# Autodesk Inventor assembly: Walls--Basement
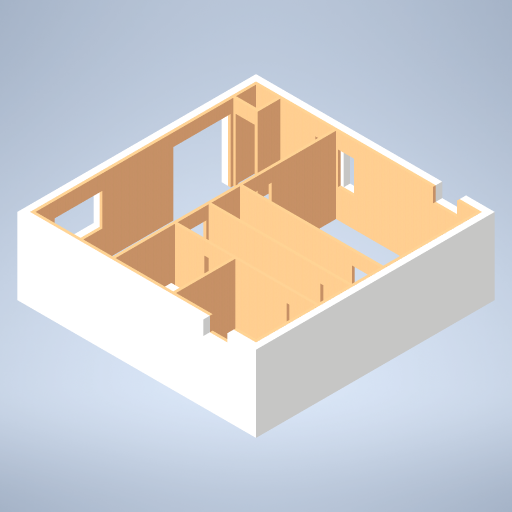
[picture p0: Inventor's stored thumbnail of the model, 512x512]
Saved by Autodesk Inventor 2024 (Build 280153000, 153)
## iProperties
Created: 2023-05-13
Part Number: Walls--Basement
Document SubType Name: Assembly
Designer: Tom
Author: Tom
## Documents named in this file (9)
- C:\Users\Tom\Documents\Tom_Levers_Public_Git_Repository\Inventor\Mobility\Basement\Finished_Basement.iam
- C:\Users\Tom\Documents\Tom_Levers_Public_Git_Repository\Inventor\Mobility\Basement\Walls--Exterior.ipt
- C:\Users\Tom\Documents\Tom_Levers_Public_Git_Repository\Inventor\Mobility\Basement\Walls--Interior.ipt
- C:\Users\Tom\Documents\Tom_Levers_Public_Git_Repository\Inventor\Mobility\Basement\Bathtub.ipt
- C:\Users\Tom\Documents\Tom_Levers_Public_Git_Repository\Inventor\Mobility\Basement\Sink--Bathroom.ipt
- C:\Users\Tom\Documents\Tom_Levers_Public_Git_Repository\Inventor\Mobility\Basement\Toilet.ipt
- C:\Users\Tom\Documents\Tom_Levers_Public_Git_Repository\Inventor\Mobility\Basement\Washer.ipt
- C:\Users\Tom\Documents\Tom_Levers_Public_Git_Repository\Inventor\Mobility\Basement\Drier.ipt
- C:\Users\Tom\Documents\Tom_Levers_Public_Git_Repository\Inventor\Mobility\Basement\Sink--Laundry.ipt
## Components (8 placed, 8 different names)
1. Walls--Exterior:1 — Mate:1, Mate:2, Flush:1, Mate:3, Flush:2, Mate:4, Mate:5, Mate:6, Flush:3, Mate:12, Flush:5, Flush:6, Flush:7
2. Walls--Interior:1 — Mate:1, Mate:2, Flush:1, Mate:3, Flush:2, Mate:4, Mate:5, Mate:6, Flush:3, Mate:8, Flush:4, Mate:9, Mate:10, Mate:11, Mate:13, Mate:19, Mate:20, Mate:21, Mate:23, Mate:24, Mate:25, Flush:8, Mate:26, Mate:27
3. Bathtub:1 — Mate:8, Flush:4, Mate:9, Mate:19, Mate:26
4. Sink--Bathroom:1 — Mate:10, Mate:11, Mate:12, Mate:14
5. Toilet:1 — Mate:13, Flush:5, Mate:14
6. Washer:1 — Mate:20, Mate:21, Flush:6
7. Drier:1 — Mate:23, Flush:7, Mate:27
8. Sink--Laundry:1 — Mate:24, Mate:25, Flush:8
## Relationships (29: Mate 21, Flush 8)
- Mate:1: Walls--Exterior:1 ↔ Walls--Interior:1
- Mate:2: Walls--Exterior:1 ↔ Walls--Interior:1
- Flush:1: Walls--Exterior:1 ↔ Walls--Interior:1
- Mate:3: Walls--Exterior:1 ↔ Walls--Interior:1
- Flush:2: Walls--Exterior:1 ↔ Walls--Interior:1
- Mate:4: Walls--Exterior:1 ↔ Walls--Interior:1
- Mate:5: Walls--Exterior:1 ↔ Walls--Interior:1
- Mate:6: Walls--Exterior:1 ↔ Walls--Interior:1
- Flush:3: Walls--Exterior:1 ↔ Walls--Interior:1
- Mate:8: Walls--Interior:1 ↔ Bathtub:1
- Flush:4: Walls--Interior:1 ↔ Bathtub:1
- Mate:9: Walls--Interior:1 ↔ Bathtub:1
- Mate:10: Walls--Interior:1 ↔ Sink--Bathroom:1
- Mate:11 (101.6 mm): Walls--Interior:1 ↔ Sink--Bathroom:1
- Mate:12 (-914.4 mm): Walls--Exterior:1 ↔ Sink--Bathroom:1
- Mate:13: Walls--Interior:1 ↔ Toilet:1
- Flush:5: Walls--Exterior:1 ↔ Toilet:1
- Mate:14 (431.8 mm): Sink--Bathroom:1 ↔ Toilet:1
- Mate:19: Walls--Interior:1 ↔ Bathtub:1
- Mate:20 (38.1 mm): Walls--Interior:1 ↔ Washer:1
- Mate:21: Walls--Interior:1 ↔ Washer:1
- Flush:6: Walls--Exterior:1 ↔ Washer:1
- Mate:23: Walls--Interior:1 ↔ Drier:1
- Flush:7: Walls--Exterior:1 ↔ Drier:1
- Mate:24: Walls--Interior:1 ↔ Sink--Laundry:1
- Mate:25 (114.3 mm): Walls--Interior:1 ↔ Sink--Laundry:1
- Flush:8: Walls--Interior:1 ↔ Sink--Laundry:1
- Mate:26: Walls--Interior:1 ↔ Bathtub:1
- Mate:27 (38.1 mm): Walls--Interior:1 ↔ Drier:1
